# Autodesk Inventor assembly: Effector_Arm_Ball
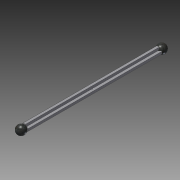
[picture p0: Inventor's stored thumbnail of the model, 180x180]
Saved by Autodesk Inventor 2014 (Build 180170000, 170)
## iProperties
Created: 2014-10-17
Part Number: Effector_Arm_Ball
Document SubType Name: Assembly
Designer: ThatOtherGuy
Author: ThatOtherGuy
## Documents named in this file (3)
- U:\Hobbies\Inventor\KosselCNC1515\Effector\Effector_Arm_Ball.iam
- U:\Hobbies\Inventor\KosselCNC1515\Joints\Joint_Ball_Bearing_12MM.ipt
- U:\Hobbies\Inventor\KosselCNC1515\Effector\Effector_Arm_Ball.ipt
## Components (4 placed, 2 different names)
1. Joint_Ball_Bearing_12MM:1 — Tangent:1, Tangent:2
2. Joint_Ball_Bearing_12MM:2 — Tangent:3, Tangent:4
3. Effector_Arm_Ball:1 — Mate:1, Mate:2, Mate:3, Tangent:1, Tangent:4
4. Effector_Arm_Ball:2 — Mate:1, Mate:2, Mate:3, Tangent:2, Tangent:3
## Relationships (7: Tangent 4, Mate 3)
- Mate:1: Effector_Arm_Ball:1 ↔ Effector_Arm_Ball:2
- Mate:2: Effector_Arm_Ball:1 ↔ Effector_Arm_Ball:2
- Mate:3: Effector_Arm_Ball:1 ↔ Effector_Arm_Ball:2
- Tangent:1: Joint_Ball_Bearing_12MM:1 ↔ Effector_Arm_Ball:1
- Tangent:2: Joint_Ball_Bearing_12MM:1 ↔ Effector_Arm_Ball:2
- Tangent:3: Joint_Ball_Bearing_12MM:2 ↔ Effector_Arm_Ball:2
- Tangent:4: Joint_Ball_Bearing_12MM:2 ↔ Effector_Arm_Ball:1
